# Autodesk Inventor assembly: Arm_left_v3
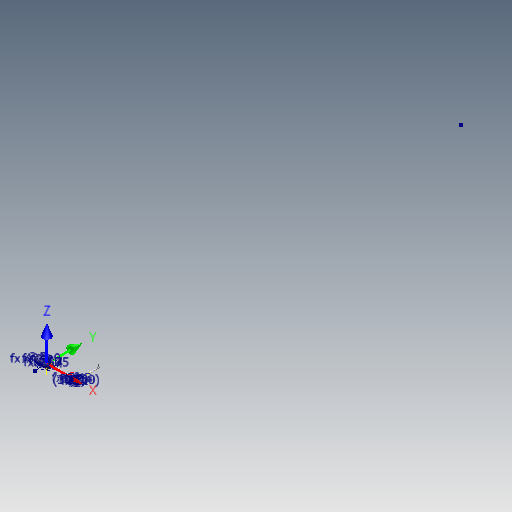
[picture p0: Inventor's stored thumbnail of the model, 512x512]
Saved by Autodesk Inventor 2021.4 (Build 254397000, 397)
## iProperties
Created: 2022-07-06
Part Number: Arm_left_v3
Material: Generisch
Document SubType Name: Assembly
Designer: alexw
Mass: 655.07 g
Surface Area: 1152.93 cm^2
Volume: 246.284 cm^3
Density: 2.65982 g/cm^3
Author: alexw
## Documents named in this file (8)
- C:\Users\alexw\Documents\Inventor\Projects\03_CurrentProjects\MasterThesis\TrainingConsol_220422\Workgroups\Workgroup\Arm_left_v3.iam
- C:\Users\alexw\Documents\Inventor\Projects\03_CurrentProjects\MasterThesis\TrainingConsol_220422\Workgroups\Workgroup\Upper_Arm_v2_Assembly.iam
- C:\Users\alexw\Documents\Inventor\Projects\03_CurrentProjects\MasterThesis\TrainingConsol_220422\Workgroups\Workgroup\Lower_Arm_v3_Assembly.iam
- C:\Users\alexw\Documents\Inventor\Projects\03_CurrentProjects\MasterThesis\TrainingConsol_220422\Workgroups\Workgroup\PTFE_Anlaufscheibe.ipt
- C:\Users\alexw\Documents\Inventor\Projects\03_CurrentProjects\MasterThesis\TrainingConsol_220422\Workgroups\Workgroup\ContentCenter\en-US\ISO 7089\ISO 7089 - 4 - 140 HV(1).ipt
- C:\Users\alexw\Documents\Inventor\Projects\03_CurrentProjects\MasterThesis\TrainingConsol_220422\Workgroups\Workgroup\ContentCenter\en-US\ISO 4017(1)\ISO 4017 - M4 x 12 - ISO.ipt
- C:\Users\alexw\Documents\Inventor\Projects\03_CurrentProjects\MasterThesis\TrainingConsol_220422\Workgroups\Workgroup\LeftArm_ShoulderJoint_Concept1_LightWeight_Assembly.iam
- C:\Users\alexw\Documents\Inventor\Projects\03_CurrentProjects\MasterThesis\TrainingConsol_220422\Workgroups\Workgroup\CounterWeights_Brass.ipt
## Components (7 placed, 7 different names)
1. LeftArm_ShoulderJoint_Concept1_LightWeight_Assembly:1 [sub-assembly] — Flush:1, Flush:2, Flush:3, Flush:14, Mate:13, Mate:14, Angle:3
2. Upper_Arm_v2_Assembly:1 [sub-assembly] — Mate:3, Mate:4, Mate:5, Mate:6, Mate:7, Mate:8, Mate:10, Mate:12, Flush:14, Mate:13, Angle:1, Angle:3
3. Lower_Arm_v3_Assembly:1 [sub-assembly] — Mate:3, Mate:4, Mate:5, Angle:1
4. PTFE_Anlaufscheibe:1 — Mate:6, Mate:7
5. ISO 7089 4:1 — Mate:8, Mate:11, Mate:12
6. ISO 4017 M4 x 12:1 — Mate:10, Mate:11
7. CounterWeights_Brass:1 — Mate:14
## Relationships (17: Mate 11, Flush 4, Angle 2)
- Flush:1: LeftArm_ShoulderJoint_Concept1_LightWeight_Assembly:1
- Flush:2: LeftArm_ShoulderJoint_Concept1_LightWeight_Assembly:1
- Flush:3: LeftArm_ShoulderJoint_Concept1_LightWeight_Assembly:1
- Mate:3: Upper_Arm_v2_Assembly:1 ↔ Lower_Arm_v3_Assembly:1
- Mate:4: Upper_Arm_v2_Assembly:1 ↔ Lower_Arm_v3_Assembly:1
- Mate:5: Upper_Arm_v2_Assembly:1 ↔ Lower_Arm_v3_Assembly:1
- Mate:6: Upper_Arm_v2_Assembly:1 ↔ PTFE_Anlaufscheibe:1
- Mate:7: Upper_Arm_v2_Assembly:1 ↔ PTFE_Anlaufscheibe:1
- Mate:8: Upper_Arm_v2_Assembly:1 ↔ ISO 7089 4:1
- Mate:10: Upper_Arm_v2_Assembly:1 ↔ ISO 4017 M4 x 12:1
- Mate:11: ISO 7089 4:1 ↔ ISO 4017 M4 x 12:1
- Mate:12: Upper_Arm_v2_Assembly:1 ↔ ISO 7089 4:1
- Flush:14: LeftArm_ShoulderJoint_Concept1_LightWeight_Assembly:1 ↔ Upper_Arm_v2_Assembly:1
- Mate:13: LeftArm_ShoulderJoint_Concept1_LightWeight_Assembly:1 ↔ Upper_Arm_v2_Assembly:1
- Mate:14: LeftArm_ShoulderJoint_Concept1_LightWeight_Assembly:1 ↔ CounterWeights_Brass:1
- Angle:1 (0 deg): Upper_Arm_v2_Assembly:1 ↔ Lower_Arm_v3_Assembly:1
- Angle:3 (0 deg): LeftArm_ShoulderJoint_Concept1_LightWeight_Assembly:1 ↔ Upper_Arm_v2_Assembly:1
